# Autodesk Inventor assembly: ShredderImperial
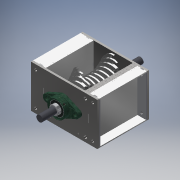
[picture p0: Inventor's stored thumbnail of the model, 180x180]
Saved by Autodesk Inventor 2018 (Build 220112000, 112)
## iProperties
Created: 2018-01-25
Part Number: ShredderImperial
Document SubType Name: Assembly
Designer: Olivier
Author: Olivier
## Documents named in this file (20)
- C:\Users\Olivier\OneDrive\Proyectos Olivier\Proyecto Shredder\Conversión Imperial\Inventor\Shredder Imperial\Autodesk Inventor 2018 files\ShredderImperial.iam
- C:\Users\Olivier\OneDrive\Proyectos Olivier\Proyecto Shredder\Conversión Imperial\Inventor\Shredder Imperial\Autodesk Inventor 2018 files\1-4inch_SidePanel_2-Parts.ipt
- C:\Users\Olivier\OneDrive\Proyectos Olivier\Proyecto Shredder\Conversión Imperial\Inventor\Shredder Imperial\Autodesk Inventor 2018 files\snr_ucfl204_0.ipt
- C:\Users\Olivier\OneDrive\Proyectos Olivier\Proyecto Shredder\Conversión Imperial\Inventor\Shredder Imperial\Autodesk Inventor 2018 files\HexBar1Inch.ipt
- C:\Users\Olivier\OneDrive\Proyectos Olivier\Proyecto Shredder\Conversión Imperial\Inventor\Shredder Imperial\Autodesk Inventor 2018 files\1-4inch_BearingSpacer_2-Parts.ipt
- C:\Users\Olivier\OneDrive\Proyectos Olivier\Proyecto Shredder\Conversión Imperial\Inventor\Shredder Imperial\Autodesk Inventor 2018 files\1-8inch_BearingSpacer_2-Parts.ipt
- C:\Users\Olivier\OneDrive\Proyectos Olivier\Proyecto Shredder\Conversión Imperial\Inventor\Shredder Imperial\Autodesk Inventor 2018 files\3-16inch_Knife1_5-Parts.ipt
- C:\Users\Olivier\OneDrive\Proyectos Olivier\Proyecto Shredder\Conversión Imperial\Inventor\Shredder Imperial\Autodesk Inventor 2018 files\3-16inch_Knife2_5-Parts.ipt
- C:\Users\Olivier\OneDrive\Proyectos Olivier\Proyecto Shredder\Conversión Imperial\Inventor\Shredder Imperial\Autodesk Inventor 2018 files\3-16inch_Knife3_4-Parts.ipt
- C:\Users\Olivier\OneDrive\Proyectos Olivier\Proyecto Shredder\Conversión Imperial\Inventor\Shredder Imperial\Autodesk Inventor 2018 files\1-4inch_KnifeSpacer_13-Parts.ipt
- C:\Users\Olivier\OneDrive\Proyectos Olivier\Proyecto Shredder\Conversión Imperial\Inventor\Shredder Imperial\Autodesk Inventor 2018 files\1-8inch_Sieve_2Parts.ipt
- C:\Users\Olivier\OneDrive\Proyectos Olivier\Proyecto Shredder\Conversión Imperial\Inventor\Shredder Imperial\Autodesk Inventor 2018 files\1-8inch_Side1_2-Parts.ipt
- C:\Users\Olivier\OneDrive\Proyectos Olivier\Proyecto Shredder\Conversión Imperial\Inventor\Shredder Imperial\Autodesk Inventor 2018 files\1-8inch_Side2_2-Parts.ipt
- C:\Users\Olivier\OneDrive\Proyectos Olivier\Proyecto Shredder\Conversión Imperial\Inventor\Shredder Imperial\Autodesk Inventor 2018 files\1-8inch_Top1_1-Part.ipt
- C:\Users\Olivier\OneDrive\Proyectos Olivier\Proyecto Shredder\Conversión Imperial\Inventor\Shredder Imperial\Autodesk Inventor 2018 files\1-8inch_Top2_1-Part.ipt
- C:\Users\Olivier\OneDrive\Proyectos Olivier\Proyecto Shredder\Conversión Imperial\Inventor\Shredder Imperial\Autodesk Inventor 2018 files\1-8inch_Bottom1_1-Part.ipt
- C:\Users\Olivier\OneDrive\Proyectos Olivier\Proyecto Shredder\Conversión Imperial\Inventor\Shredder Imperial\Autodesk Inventor 2018 files\1-8inch_Bottom2_1-Part.ipt
- C:\Users\Olivier\OneDrive\Proyectos Olivier\Proyecto Shredder\Conversión Imperial\Inventor\Shredder Imperial\Autodesk Inventor 2018 files\1-4inch_FixedKnifeSmall_14-Parts.ipt
- C:\Users\Olivier\OneDrive\Proyectos Olivier\Proyecto Shredder\Conversión Imperial\Inventor\Shredder Imperial\Autodesk Inventor 2018 files\3-16inch_FixedKnifeBig_13-Parts.ipt
- C:\Users\Olivier\OneDrive\Proyectos Olivier\Proyecto Shredder\Conversión Imperial\Inventor\Shredder Imperial\Autodesk Inventor 2018 files\1-8inch_Middle_2-Parts.ipt
## Components (75 placed, 19 different names)
1. 1-8inch_Middle_2-Parts:1 — Flush:18, Mate:233, Mate:234, Flush:20, Flush:21
2. 1-8inch_Middle_2-Parts:2 — Mate:225, Flush:14, Mate:226
3. 1-4inch_SidePanel_2-Parts:1 — Insert:1, Insert:2, Mate:96, Mate:97, Mate:120, Mate:121, Mate:123, Mate:215, Flush:13, Mate:222, Mate:223, Mate:224, Flush:15, Mate:230, Mate:231, Mate:232, Mate:233, Mate:235, Mate:236
4. 1-4inch_SidePanel_2-Parts:2 — Mate:91, Mate:92, Mate:93, Mate:94, Mate:95, Mate:203, Mate:204, Mate:207, Mate:218, Mate:219, Mate:220, Mate:225, Flush:14, Mate:227, Mate:228, Mate:229, Flush:16, Flush:18, Flush:19
5. 3-16inch_FixedKnifeBig_13-Parts:1 — Mate:122, Mate:124, Mate:125, Mate:126, Mate:127, Mate:128
6. 3-16inch_FixedKnifeBig_13-Parts:2 — Mate:129, Mate:130, Mate:131, Mate:132, Mate:133, Mate:134
7. 3-16inch_FixedKnifeBig_13-Parts:3 — Mate:135, Mate:136, Mate:137, Mate:138, Mate:139, Mate:140
8. 3-16inch_FixedKnifeBig_13-Parts:4 — Mate:141, Mate:142, Mate:143, Mate:144, Mate:145, Mate:146
9. 3-16inch_FixedKnifeBig_13-Parts:5 — Mate:147, Mate:148, Mate:149, Mate:150, Mate:151, Mate:152
10. 3-16inch_FixedKnifeBig_13-Parts:6 — Mate:153, Mate:154, Mate:155, Mate:156, Mate:157, Mate:158
11. 3-16inch_FixedKnifeBig_13-Parts:7 — Mate:159, Mate:160, Mate:161, Mate:162, Mate:163, Mate:164
12. 3-16inch_FixedKnifeBig_13-Parts:8 — Mate:165, Mate:166, Mate:167, Mate:168, Mate:169, Mate:170
13. 3-16inch_FixedKnifeBig_13-Parts:9 — Mate:171, Mate:172, Mate:173, Mate:174, Mate:175, Mate:176
14. 3-16inch_FixedKnifeBig_13-Parts:10 — Mate:177, Mate:178, Mate:179, Mate:180, Mate:181, Mate:182
15. 3-16inch_FixedKnifeBig_13-Parts:11 — Mate:183, Mate:184, Mate:185, Mate:186, Mate:187, Mate:188
16. 3-16inch_FixedKnifeBig_13-Parts:12 — Mate:189, Mate:190, Mate:191, Mate:192, Mate:193, Mate:194
17. 3-16inch_FixedKnifeBig_13-Parts:13 — Mate:195, Mate:196, Mate:197, Mate:198, Mate:199, Mate:200
18. 1-4inch_FixedKnifeSmall_14-Parts:1 — Mate:120, Mate:121, Mate:122, Mate:123, Mate:124, Mate:125, Mate:226
19. 1-4inch_FixedKnifeSmall_14-Parts:2 — Mate:126, Mate:127, Mate:128, Mate:129, Mate:130, Mate:131
20. 1-4inch_FixedKnifeSmall_14-Parts:3 — Mate:132, Mate:133, Mate:134, Mate:135, Mate:136, Mate:137
21. 1-4inch_FixedKnifeSmall_14-Parts:4 — Mate:138, Mate:139, Mate:140, Mate:141, Mate:142, Mate:143
22. 1-4inch_FixedKnifeSmall_14-Parts:5 — Mate:144, Mate:145, Mate:146, Mate:147, Mate:148, Mate:149
23. 1-4inch_FixedKnifeSmall_14-Parts:6 — Mate:150, Mate:151, Mate:152, Mate:153, Mate:154, Mate:155
24. 1-4inch_FixedKnifeSmall_14-Parts:7 — Mate:156, Mate:157, Mate:158, Mate:159, Mate:160, Mate:161
25. 1-4inch_FixedKnifeSmall_14-Parts:8 — Mate:162, Mate:163, Mate:164, Mate:165, Mate:166, Mate:167
26. 1-4inch_FixedKnifeSmall_14-Parts:9 — Mate:168, Mate:169, Mate:170, Mate:171, Mate:172, Mate:173
27. 1-4inch_FixedKnifeSmall_14-Parts:10 — Mate:174, Mate:175, Mate:176, Mate:177, Mate:178, Mate:179
28. 1-4inch_FixedKnifeSmall_14-Parts:11 — Mate:180, Mate:181, Mate:182, Mate:183, Mate:184, Mate:185
29. 1-4inch_FixedKnifeSmall_14-Parts:12 — Mate:186, Mate:187, Mate:188, Mate:189, Mate:190, Mate:191
30. 1-4inch_FixedKnifeSmall_14-Parts:13 — Mate:192, Mate:193, Mate:194, Mate:195, Mate:196, Mate:197
31. 1-4inch_FixedKnifeSmall_14-Parts:14 — Mate:198, Mate:199, Mate:200, Mate:203, Mate:204
32. HexBar1Inch:1 — Insert:3, Insert:4, Mate:5, Mate:6, Mate:7, Mate:9, Mate:10, Mate:11, Mate:12, Mate:13, Mate:15, Mate:16, Mate:17, Mate:18, Mate:21, Mate:22, Mate:23, Mate:24, Mate:27, Mate:28, Mate:30, Mate:31, Mate:33, Mate:34, Mate:36, Mate:37, Mate:39, Mate:40, Mate:42, Mate:43, Mate:45, Mate:46, Mate:48, Mate:49, Mate:51, Mate:52, Mate:54, Mate:55, Mate:57, Mate:58, Mate:60, Mate:61, Mate:63, Mate:64, Mate:66, Mate:67, Mate:69, Mate:70, Mate:71, Mate:72, Mate:75, Mate:76, Mate:78, Mate:79, Mate:80, Mate:82, Mate:83, Mate:85, Mate:86
33. snr_ucfl204_0:2 — Mate:91, Mate:92, Mate:93
34. snr_ucfl204_0:1 — Insert:1, Insert:2, Insert:7
35. 3-16inch_Knife1_5-Parts:1 — Mate:5, Mate:6, Mate:7, Mate:8
36. 3-16inch_Knife1_5-Parts:2 — Mate:21, Mate:22, Mate:26, Mate:29
37. 3-16inch_Knife1_5-Parts:3 — Mate:42, Mate:43, Mate:44, Mate:47
38. 3-16inch_Knife1_5-Parts:4 — Mate:60, Mate:61, Mate:62, Mate:65
39. 3-16inch_Knife1_5-Parts:5 — Mate:78, Mate:79, Mate:80, Mate:81, Mate:84
40. 3-16inch_Knife2_5-Parts:1 — Mate:12, Mate:13, Mate:14, Mate:19
41. 3-16inch_Knife2_5-Parts:2 — Mate:30, Mate:31, Mate:32, Mate:35
42. 3-16inch_Knife2_5-Parts:3 — Mate:48, Mate:49, Mate:50, Mate:53
43. 3-16inch_Knife2_5-Parts:4 — Mate:66, Mate:67, Mate:68, Mate:73
44. 3-16inch_Knife2_5-Parts:5 — Mate:85, Mate:86, Mate:87
45. 3-16inch_Knife3_4-Parts:1 — Mate:15, Mate:16, Mate:20, Mate:25
46. 3-16inch_Knife3_4-Parts:2 — Mate:36, Mate:37, Mate:38, Mate:41
47. 3-16inch_Knife3_4-Parts:3 — Mate:54, Mate:55, Mate:56, Mate:59
48. 3-16inch_Knife3_4-Parts:4 — Mate:69, Mate:70, Mate:74, Mate:77
49. 1-8inch_BearingSpacer_2-Parts:1 — Insert:3, Insert:5
50. 1-8inch_BearingSpacer_2-Parts:2 — Insert:4, Insert:6
51. 1-4inch_BearingSpacer_2-Parts:1 — Insert:5, Insert:7
52. 1-4inch_BearingSpacer_2-Parts:2 — Insert:6
53. 1-4inch_KnifeSpacer_13-Parts:1 — Mate:8, Mate:9, Mate:10, Mate:11, Mate:14
54. 1-4inch_KnifeSpacer_13-Parts:2 — Mate:17, Mate:18, Mate:19, Mate:20
55. 1-4inch_KnifeSpacer_13-Parts:3 — Mate:23, Mate:24, Mate:25, Mate:26
56. 1-4inch_KnifeSpacer_13-Parts:4 — Mate:27, Mate:28, Mate:29, Mate:32
57. 1-4inch_KnifeSpacer_13-Parts:5 — Mate:33, Mate:34, Mate:35, Mate:38
58. 1-4inch_KnifeSpacer_13-Parts:6 — Mate:39, Mate:40, Mate:41, Mate:44
59. 1-4inch_KnifeSpacer_13-Parts:7 — Mate:45, Mate:46, Mate:47, Mate:50
60. 1-4inch_KnifeSpacer_13-Parts:8 — Mate:51, Mate:52, Mate:53, Mate:56
61. 1-4inch_KnifeSpacer_13-Parts:9 — Mate:57, Mate:58, Mate:59, Mate:62
62. 1-4inch_KnifeSpacer_13-Parts:10 — Mate:63, Mate:64, Mate:65, Mate:68
63. 1-4inch_KnifeSpacer_13-Parts:11 — Mate:71, Mate:72, Mate:73, Mate:74
64. 1-4inch_KnifeSpacer_13-Parts:12 — Mate:75, Mate:76, Mate:77, Mate:81
65. 1-4inch_KnifeSpacer_13-Parts:13 — Mate:82, Mate:83, Mate:84, Mate:87
66. 1-8inch_Sieve_2Parts:2 — Mate:94, Mate:95
67. 1-8inch_Sieve_2Parts:1 — Mate:96, Mate:97
68. 1-8inch_Side1_2-Parts:1 — Mate:218, Mate:219, Mate:220
69. 1-8inch_Side1_2-Parts:2 — Mate:222, Mate:223, Mate:224
70. 1-8inch_Bottom1_1-Part:1 — Mate:215, Flush:13, Flush:15
71. 1-8inch_Top1_1-Part:1 — Mate:207
72. 1-8inch_Side2_2-Parts:1 — Mate:227, Mate:228, Mate:229
73. 1-8inch_Side2_2-Parts:2 — Mate:230, Mate:231, Mate:232, Mate:234
74. 1-8inch_Bottom2_1-Part:1 — Flush:16, Flush:21, Mate:236
75. 1-8inch_Top2_1-Part:1 — Flush:19, Mate:235, Flush:20
## Relationships (208: Mate 193, Flush 8, Insert 7)
- Insert:1: 1-4inch_SidePanel_2-Parts:1 ↔ snr_ucfl204_0:1
- Insert:2: 1-4inch_SidePanel_2-Parts:1 ↔ snr_ucfl204_0:1
- Insert:3: HexBar1Inch:1 ↔ 1-8inch_BearingSpacer_2-Parts:1
- Insert:4: HexBar1Inch:1 ↔ 1-8inch_BearingSpacer_2-Parts:2
- Insert:5: 1-8inch_BearingSpacer_2-Parts:1 ↔ 1-4inch_BearingSpacer_2-Parts:1
- Insert:6: 1-8inch_BearingSpacer_2-Parts:2 ↔ 1-4inch_BearingSpacer_2-Parts:2
- Insert:7: snr_ucfl204_0:1 ↔ 1-4inch_BearingSpacer_2-Parts:1
- Mate:5: HexBar1Inch:1 ↔ 3-16inch_Knife1_5-Parts:1
- Mate:6: HexBar1Inch:1 ↔ 3-16inch_Knife1_5-Parts:1
- Mate:7: HexBar1Inch:1 ↔ 3-16inch_Knife1_5-Parts:1
- Mate:8: 3-16inch_Knife1_5-Parts:1 ↔ 1-4inch_KnifeSpacer_13-Parts:1
- Mate:9: HexBar1Inch:1 ↔ 1-4inch_KnifeSpacer_13-Parts:1
- Mate:10: HexBar1Inch:1 ↔ 1-4inch_KnifeSpacer_13-Parts:1
- Mate:11: HexBar1Inch:1 ↔ 1-4inch_KnifeSpacer_13-Parts:1
- Mate:12: HexBar1Inch:1 ↔ 3-16inch_Knife2_5-Parts:1
- Mate:13: HexBar1Inch:1 ↔ 3-16inch_Knife2_5-Parts:1
- Mate:14: 3-16inch_Knife2_5-Parts:1 ↔ 1-4inch_KnifeSpacer_13-Parts:1
- Mate:15: HexBar1Inch:1 ↔ 3-16inch_Knife3_4-Parts:1
- Mate:16: HexBar1Inch:1 ↔ 3-16inch_Knife3_4-Parts:1
- Mate:17: HexBar1Inch:1 ↔ 1-4inch_KnifeSpacer_13-Parts:2
- Mate:18: HexBar1Inch:1 ↔ 1-4inch_KnifeSpacer_13-Parts:2
- Mate:19: 3-16inch_Knife2_5-Parts:1 ↔ 1-4inch_KnifeSpacer_13-Parts:2
- Mate:20: 3-16inch_Knife3_4-Parts:1 ↔ 1-4inch_KnifeSpacer_13-Parts:2
- Mate:21: HexBar1Inch:1 ↔ 3-16inch_Knife1_5-Parts:2
- Mate:22: HexBar1Inch:1 ↔ 3-16inch_Knife1_5-Parts:2
- Mate:23: HexBar1Inch:1 ↔ 1-4inch_KnifeSpacer_13-Parts:3
- Mate:24: HexBar1Inch:1 ↔ 1-4inch_KnifeSpacer_13-Parts:3
- Mate:25: 3-16inch_Knife3_4-Parts:1 ↔ 1-4inch_KnifeSpacer_13-Parts:3
- Mate:26: 3-16inch_Knife1_5-Parts:2 ↔ 1-4inch_KnifeSpacer_13-Parts:3
- Mate:27: HexBar1Inch:1 ↔ 1-4inch_KnifeSpacer_13-Parts:4
- Mate:28: HexBar1Inch:1 ↔ 1-4inch_KnifeSpacer_13-Parts:4
- Mate:29: 3-16inch_Knife1_5-Parts:2 ↔ 1-4inch_KnifeSpacer_13-Parts:4
- Mate:30: HexBar1Inch:1 ↔ 3-16inch_Knife2_5-Parts:2
- Mate:31: HexBar1Inch:1 ↔ 3-16inch_Knife2_5-Parts:2
- Mate:32: 3-16inch_Knife2_5-Parts:2 ↔ 1-4inch_KnifeSpacer_13-Parts:4
- Mate:33: HexBar1Inch:1 ↔ 1-4inch_KnifeSpacer_13-Parts:5
- Mate:34: HexBar1Inch:1 ↔ 1-4inch_KnifeSpacer_13-Parts:5
- Mate:35: 3-16inch_Knife2_5-Parts:2 ↔ 1-4inch_KnifeSpacer_13-Parts:5
- Mate:36: HexBar1Inch:1 ↔ 3-16inch_Knife3_4-Parts:2
- Mate:37: HexBar1Inch:1 ↔ 3-16inch_Knife3_4-Parts:2
- Mate:38: 3-16inch_Knife3_4-Parts:2 ↔ 1-4inch_KnifeSpacer_13-Parts:5
- Mate:39: HexBar1Inch:1 ↔ 1-4inch_KnifeSpacer_13-Parts:6
- Mate:40: HexBar1Inch:1 ↔ 1-4inch_KnifeSpacer_13-Parts:6
- Mate:41: 3-16inch_Knife3_4-Parts:2 ↔ 1-4inch_KnifeSpacer_13-Parts:6
- Mate:42: HexBar1Inch:1 ↔ 3-16inch_Knife1_5-Parts:3
- Mate:43: HexBar1Inch:1 ↔ 3-16inch_Knife1_5-Parts:3
- Mate:44: 3-16inch_Knife1_5-Parts:3 ↔ 1-4inch_KnifeSpacer_13-Parts:6
- Mate:45: HexBar1Inch:1 ↔ 1-4inch_KnifeSpacer_13-Parts:7
- Mate:46: HexBar1Inch:1 ↔ 1-4inch_KnifeSpacer_13-Parts:7
- Mate:47: 3-16inch_Knife1_5-Parts:3 ↔ 1-4inch_KnifeSpacer_13-Parts:7
- Mate:48: HexBar1Inch:1 ↔ 3-16inch_Knife2_5-Parts:3
- Mate:49: HexBar1Inch:1 ↔ 3-16inch_Knife2_5-Parts:3
- Mate:50: 3-16inch_Knife2_5-Parts:3 ↔ 1-4inch_KnifeSpacer_13-Parts:7
- Mate:51: HexBar1Inch:1 ↔ 1-4inch_KnifeSpacer_13-Parts:8
- Mate:52: HexBar1Inch:1 ↔ 1-4inch_KnifeSpacer_13-Parts:8
- Mate:53: 3-16inch_Knife2_5-Parts:3 ↔ 1-4inch_KnifeSpacer_13-Parts:8
- Mate:54: HexBar1Inch:1 ↔ 3-16inch_Knife3_4-Parts:3
- Mate:55: HexBar1Inch:1 ↔ 3-16inch_Knife3_4-Parts:3
- Mate:56: 3-16inch_Knife3_4-Parts:3 ↔ 1-4inch_KnifeSpacer_13-Parts:8
- Mate:57: HexBar1Inch:1 ↔ 1-4inch_KnifeSpacer_13-Parts:9
- Mate:58: HexBar1Inch:1 ↔ 1-4inch_KnifeSpacer_13-Parts:9
- Mate:59: 3-16inch_Knife3_4-Parts:3 ↔ 1-4inch_KnifeSpacer_13-Parts:9
- Mate:60: HexBar1Inch:1 ↔ 3-16inch_Knife1_5-Parts:4
- Mate:61: HexBar1Inch:1 ↔ 3-16inch_Knife1_5-Parts:4
- Mate:62: 3-16inch_Knife1_5-Parts:4 ↔ 1-4inch_KnifeSpacer_13-Parts:9
- Mate:63: HexBar1Inch:1 ↔ 1-4inch_KnifeSpacer_13-Parts:10
- Mate:64: HexBar1Inch:1 ↔ 1-4inch_KnifeSpacer_13-Parts:10
- Mate:65: 3-16inch_Knife1_5-Parts:4 ↔ 1-4inch_KnifeSpacer_13-Parts:10
- Mate:66: HexBar1Inch:1 ↔ 3-16inch_Knife2_5-Parts:4
- Mate:67: HexBar1Inch:1 ↔ 3-16inch_Knife2_5-Parts:4
- Mate:68: 3-16inch_Knife2_5-Parts:4 ↔ 1-4inch_KnifeSpacer_13-Parts:10
- Mate:69: HexBar1Inch:1 ↔ 3-16inch_Knife3_4-Parts:4
- Mate:70: HexBar1Inch:1 ↔ 3-16inch_Knife3_4-Parts:4
- Mate:71: HexBar1Inch:1 ↔ 1-4inch_KnifeSpacer_13-Parts:11
- Mate:72: HexBar1Inch:1 ↔ 1-4inch_KnifeSpacer_13-Parts:11
- Mate:73: 3-16inch_Knife2_5-Parts:4 ↔ 1-4inch_KnifeSpacer_13-Parts:11
- Mate:74: 3-16inch_Knife3_4-Parts:4 ↔ 1-4inch_KnifeSpacer_13-Parts:11
- Mate:75: HexBar1Inch:1 ↔ 1-4inch_KnifeSpacer_13-Parts:12
- Mate:76: HexBar1Inch:1 ↔ 1-4inch_KnifeSpacer_13-Parts:12
- Mate:77: 3-16inch_Knife3_4-Parts:4 ↔ 1-4inch_KnifeSpacer_13-Parts:12
- Mate:78: HexBar1Inch:1 ↔ 3-16inch_Knife1_5-Parts:5
- Mate:79: HexBar1Inch:1 ↔ 3-16inch_Knife1_5-Parts:5
- Mate:80: HexBar1Inch:1 ↔ 3-16inch_Knife1_5-Parts:5
- Mate:81: 3-16inch_Knife1_5-Parts:5 ↔ 1-4inch_KnifeSpacer_13-Parts:12
- Mate:82: HexBar1Inch:1 ↔ 1-4inch_KnifeSpacer_13-Parts:13
- Mate:83: HexBar1Inch:1 ↔ 1-4inch_KnifeSpacer_13-Parts:13
- Mate:84: 3-16inch_Knife1_5-Parts:5 ↔ 1-4inch_KnifeSpacer_13-Parts:13
- Mate:85: HexBar1Inch:1 ↔ 3-16inch_Knife2_5-Parts:5
- Mate:86: HexBar1Inch:1 ↔ 3-16inch_Knife2_5-Parts:5
- Mate:87: 3-16inch_Knife2_5-Parts:5 ↔ 1-4inch_KnifeSpacer_13-Parts:13
- Mate:91: 1-4inch_SidePanel_2-Parts:2 ↔ snr_ucfl204_0:2
- Mate:92: 1-4inch_SidePanel_2-Parts:2 ↔ snr_ucfl204_0:2
- Mate:93: 1-4inch_SidePanel_2-Parts:2 ↔ snr_ucfl204_0:2
- Mate:94: 1-4inch_SidePanel_2-Parts:2 ↔ 1-8inch_Sieve_2Parts:2
- Mate:95: 1-4inch_SidePanel_2-Parts:2 ↔ 1-8inch_Sieve_2Parts:2
- Mate:96: 1-4inch_SidePanel_2-Parts:1 ↔ 1-8inch_Sieve_2Parts:1
- Mate:97: 1-4inch_SidePanel_2-Parts:1 ↔ 1-8inch_Sieve_2Parts:1
- Mate:120: 1-4inch_SidePanel_2-Parts:1 ↔ 1-4inch_FixedKnifeSmall_14-Parts:1
- Mate:121: 1-4inch_SidePanel_2-Parts:1 ↔ 1-4inch_FixedKnifeSmall_14-Parts:1
- Mate:122: 3-16inch_FixedKnifeBig_13-Parts:1 ↔ 1-4inch_FixedKnifeSmall_14-Parts:1
- Mate:123: 1-4inch_SidePanel_2-Parts:1 ↔ 1-4inch_FixedKnifeSmall_14-Parts:1
- Mate:124: 3-16inch_FixedKnifeBig_13-Parts:1 ↔ 1-4inch_FixedKnifeSmall_14-Parts:1
- Mate:125: 3-16inch_FixedKnifeBig_13-Parts:1 ↔ 1-4inch_FixedKnifeSmall_14-Parts:1
- Mate:126: 3-16inch_FixedKnifeBig_13-Parts:1 ↔ 1-4inch_FixedKnifeSmall_14-Parts:2
- Mate:127: 3-16inch_FixedKnifeBig_13-Parts:1 ↔ 1-4inch_FixedKnifeSmall_14-Parts:2
- Mate:128: 3-16inch_FixedKnifeBig_13-Parts:1 ↔ 1-4inch_FixedKnifeSmall_14-Parts:2
- Mate:129: 3-16inch_FixedKnifeBig_13-Parts:2 ↔ 1-4inch_FixedKnifeSmall_14-Parts:2
- Mate:130: 3-16inch_FixedKnifeBig_13-Parts:2 ↔ 1-4inch_FixedKnifeSmall_14-Parts:2
- Mate:131: 3-16inch_FixedKnifeBig_13-Parts:2 ↔ 1-4inch_FixedKnifeSmall_14-Parts:2
- Mate:132: 3-16inch_FixedKnifeBig_13-Parts:2 ↔ 1-4inch_FixedKnifeSmall_14-Parts:3
- Mate:133: 3-16inch_FixedKnifeBig_13-Parts:2 ↔ 1-4inch_FixedKnifeSmall_14-Parts:3
- Mate:134: 3-16inch_FixedKnifeBig_13-Parts:2 ↔ 1-4inch_FixedKnifeSmall_14-Parts:3
- Mate:135: 3-16inch_FixedKnifeBig_13-Parts:3 ↔ 1-4inch_FixedKnifeSmall_14-Parts:3
- Mate:136: 3-16inch_FixedKnifeBig_13-Parts:3 ↔ 1-4inch_FixedKnifeSmall_14-Parts:3
- Mate:137: 3-16inch_FixedKnifeBig_13-Parts:3 ↔ 1-4inch_FixedKnifeSmall_14-Parts:3
- Mate:138: 3-16inch_FixedKnifeBig_13-Parts:3 ↔ 1-4inch_FixedKnifeSmall_14-Parts:4
- Mate:139: 3-16inch_FixedKnifeBig_13-Parts:3 ↔ 1-4inch_FixedKnifeSmall_14-Parts:4
- Mate:140: 3-16inch_FixedKnifeBig_13-Parts:3 ↔ 1-4inch_FixedKnifeSmall_14-Parts:4
- Mate:141: 3-16inch_FixedKnifeBig_13-Parts:4 ↔ 1-4inch_FixedKnifeSmall_14-Parts:4
- Mate:142: 3-16inch_FixedKnifeBig_13-Parts:4 ↔ 1-4inch_FixedKnifeSmall_14-Parts:4
- Mate:143: 3-16inch_FixedKnifeBig_13-Parts:4 ↔ 1-4inch_FixedKnifeSmall_14-Parts:4
- Mate:144: 3-16inch_FixedKnifeBig_13-Parts:4 ↔ 1-4inch_FixedKnifeSmall_14-Parts:5
- Mate:145: 3-16inch_FixedKnifeBig_13-Parts:4 ↔ 1-4inch_FixedKnifeSmall_14-Parts:5
- Mate:146: 3-16inch_FixedKnifeBig_13-Parts:4 ↔ 1-4inch_FixedKnifeSmall_14-Parts:5
- Mate:147: 3-16inch_FixedKnifeBig_13-Parts:5 ↔ 1-4inch_FixedKnifeSmall_14-Parts:5
- Mate:148: 3-16inch_FixedKnifeBig_13-Parts:5 ↔ 1-4inch_FixedKnifeSmall_14-Parts:5
- Mate:149: 3-16inch_FixedKnifeBig_13-Parts:5 ↔ 1-4inch_FixedKnifeSmall_14-Parts:5
- Mate:150: 3-16inch_FixedKnifeBig_13-Parts:5 ↔ 1-4inch_FixedKnifeSmall_14-Parts:6
- Mate:151: 3-16inch_FixedKnifeBig_13-Parts:5 ↔ 1-4inch_FixedKnifeSmall_14-Parts:6
- Mate:152: 3-16inch_FixedKnifeBig_13-Parts:5 ↔ 1-4inch_FixedKnifeSmall_14-Parts:6
- Mate:153: 3-16inch_FixedKnifeBig_13-Parts:6 ↔ 1-4inch_FixedKnifeSmall_14-Parts:6
- Mate:154: 3-16inch_FixedKnifeBig_13-Parts:6 ↔ 1-4inch_FixedKnifeSmall_14-Parts:6
- Mate:155: 3-16inch_FixedKnifeBig_13-Parts:6 ↔ 1-4inch_FixedKnifeSmall_14-Parts:6
- Mate:156: 3-16inch_FixedKnifeBig_13-Parts:6 ↔ 1-4inch_FixedKnifeSmall_14-Parts:7
- Mate:157: 3-16inch_FixedKnifeBig_13-Parts:6 ↔ 1-4inch_FixedKnifeSmall_14-Parts:7
- Mate:158: 3-16inch_FixedKnifeBig_13-Parts:6 ↔ 1-4inch_FixedKnifeSmall_14-Parts:7
- Mate:159: 3-16inch_FixedKnifeBig_13-Parts:7 ↔ 1-4inch_FixedKnifeSmall_14-Parts:7
- Mate:160: 3-16inch_FixedKnifeBig_13-Parts:7 ↔ 1-4inch_FixedKnifeSmall_14-Parts:7
- Mate:161: 3-16inch_FixedKnifeBig_13-Parts:7 ↔ 1-4inch_FixedKnifeSmall_14-Parts:7
- Mate:162: 3-16inch_FixedKnifeBig_13-Parts:7 ↔ 1-4inch_FixedKnifeSmall_14-Parts:8
- Mate:163: 3-16inch_FixedKnifeBig_13-Parts:7 ↔ 1-4inch_FixedKnifeSmall_14-Parts:8
- Mate:164: 3-16inch_FixedKnifeBig_13-Parts:7 ↔ 1-4inch_FixedKnifeSmall_14-Parts:8
- Mate:165: 3-16inch_FixedKnifeBig_13-Parts:8 ↔ 1-4inch_FixedKnifeSmall_14-Parts:8
- Mate:166: 3-16inch_FixedKnifeBig_13-Parts:8 ↔ 1-4inch_FixedKnifeSmall_14-Parts:8
- Mate:167: 3-16inch_FixedKnifeBig_13-Parts:8 ↔ 1-4inch_FixedKnifeSmall_14-Parts:8
- Mate:168: 3-16inch_FixedKnifeBig_13-Parts:8 ↔ 1-4inch_FixedKnifeSmall_14-Parts:9
- Mate:169: 3-16inch_FixedKnifeBig_13-Parts:8 ↔ 1-4inch_FixedKnifeSmall_14-Parts:9
- Mate:170: 3-16inch_FixedKnifeBig_13-Parts:8 ↔ 1-4inch_FixedKnifeSmall_14-Parts:9
- Mate:171: 3-16inch_FixedKnifeBig_13-Parts:9 ↔ 1-4inch_FixedKnifeSmall_14-Parts:9
- Mate:172: 3-16inch_FixedKnifeBig_13-Parts:9 ↔ 1-4inch_FixedKnifeSmall_14-Parts:9
- Mate:173: 3-16inch_FixedKnifeBig_13-Parts:9 ↔ 1-4inch_FixedKnifeSmall_14-Parts:9
- Mate:174: 3-16inch_FixedKnifeBig_13-Parts:9 ↔ 1-4inch_FixedKnifeSmall_14-Parts:10
- Mate:175: 3-16inch_FixedKnifeBig_13-Parts:9 ↔ 1-4inch_FixedKnifeSmall_14-Parts:10
- Mate:176: 3-16inch_FixedKnifeBig_13-Parts:9 ↔ 1-4inch_FixedKnifeSmall_14-Parts:10
- Mate:177: 3-16inch_FixedKnifeBig_13-Parts:10 ↔ 1-4inch_FixedKnifeSmall_14-Parts:10
- Mate:178: 3-16inch_FixedKnifeBig_13-Parts:10 ↔ 1-4inch_FixedKnifeSmall_14-Parts:10
- Mate:179: 3-16inch_FixedKnifeBig_13-Parts:10 ↔ 1-4inch_FixedKnifeSmall_14-Parts:10
- Mate:180: 3-16inch_FixedKnifeBig_13-Parts:10 ↔ 1-4inch_FixedKnifeSmall_14-Parts:11
- Mate:181: 3-16inch_FixedKnifeBig_13-Parts:10 ↔ 1-4inch_FixedKnifeSmall_14-Parts:11
- Mate:182: 3-16inch_FixedKnifeBig_13-Parts:10 ↔ 1-4inch_FixedKnifeSmall_14-Parts:11
- Mate:183: 3-16inch_FixedKnifeBig_13-Parts:11 ↔ 1-4inch_FixedKnifeSmall_14-Parts:11
- Mate:184: 3-16inch_FixedKnifeBig_13-Parts:11 ↔ 1-4inch_FixedKnifeSmall_14-Parts:11
- Mate:185: 3-16inch_FixedKnifeBig_13-Parts:11 ↔ 1-4inch_FixedKnifeSmall_14-Parts:11
- Mate:186: 3-16inch_FixedKnifeBig_13-Parts:11 ↔ 1-4inch_FixedKnifeSmall_14-Parts:12
- Mate:187: 3-16inch_FixedKnifeBig_13-Parts:11 ↔ 1-4inch_FixedKnifeSmall_14-Parts:12
- Mate:188: 3-16inch_FixedKnifeBig_13-Parts:11 ↔ 1-4inch_FixedKnifeSmall_14-Parts:12
- Mate:189: 3-16inch_FixedKnifeBig_13-Parts:12 ↔ 1-4inch_FixedKnifeSmall_14-Parts:12
- Mate:190: 3-16inch_FixedKnifeBig_13-Parts:12 ↔ 1-4inch_FixedKnifeSmall_14-Parts:12
- Mate:191: 3-16inch_FixedKnifeBig_13-Parts:12 ↔ 1-4inch_FixedKnifeSmall_14-Parts:12
- Mate:192: 3-16inch_FixedKnifeBig_13-Parts:12 ↔ 1-4inch_FixedKnifeSmall_14-Parts:13
- Mate:193: 3-16inch_FixedKnifeBig_13-Parts:12 ↔ 1-4inch_FixedKnifeSmall_14-Parts:13
- Mate:194: 3-16inch_FixedKnifeBig_13-Parts:12 ↔ 1-4inch_FixedKnifeSmall_14-Parts:13
- Mate:195: 3-16inch_FixedKnifeBig_13-Parts:13 ↔ 1-4inch_FixedKnifeSmall_14-Parts:13
- Mate:196: 3-16inch_FixedKnifeBig_13-Parts:13 ↔ 1-4inch_FixedKnifeSmall_14-Parts:13
- Mate:197: 3-16inch_FixedKnifeBig_13-Parts:13 ↔ 1-4inch_FixedKnifeSmall_14-Parts:13
- Mate:198: 3-16inch_FixedKnifeBig_13-Parts:13 ↔ 1-4inch_FixedKnifeSmall_14-Parts:14
- Mate:199: 3-16inch_FixedKnifeBig_13-Parts:13 ↔ 1-4inch_FixedKnifeSmall_14-Parts:14
- Mate:200: 3-16inch_FixedKnifeBig_13-Parts:13 ↔ 1-4inch_FixedKnifeSmall_14-Parts:14
- Mate:203: 1-4inch_SidePanel_2-Parts:2 ↔ 1-4inch_FixedKnifeSmall_14-Parts:14
- Mate:204: 1-4inch_SidePanel_2-Parts:2 ↔ 1-4inch_FixedKnifeSmall_14-Parts:14
- Mate:207: 1-4inch_SidePanel_2-Parts:2 ↔ 1-8inch_Top1_1-Part:1
- Mate:215: 1-4inch_SidePanel_2-Parts:1 ↔ 1-8inch_Bottom1_1-Part:1
- Flush:13: 1-4inch_SidePanel_2-Parts:1 ↔ 1-8inch_Bottom1_1-Part:1
- Mate:218: 1-4inch_SidePanel_2-Parts:2 ↔ 1-8inch_Side1_2-Parts:1
- Mate:219: 1-4inch_SidePanel_2-Parts:2 ↔ 1-8inch_Side1_2-Parts:1
- Mate:220: 1-4inch_SidePanel_2-Parts:2 ↔ 1-8inch_Side1_2-Parts:1
- Mate:222: 1-4inch_SidePanel_2-Parts:1 ↔ 1-8inch_Side1_2-Parts:2
- Mate:223: 1-4inch_SidePanel_2-Parts:1 ↔ 1-8inch_Side1_2-Parts:2
- Mate:224: 1-4inch_SidePanel_2-Parts:1 ↔ 1-8inch_Side1_2-Parts:2
- Mate:225: 1-8inch_Middle_2-Parts:2 ↔ 1-4inch_SidePanel_2-Parts:2
- Flush:14: 1-8inch_Middle_2-Parts:2 ↔ 1-4inch_SidePanel_2-Parts:2
- Mate:226: 1-8inch_Middle_2-Parts:2 ↔ 1-4inch_FixedKnifeSmall_14-Parts:1
- Flush:15: 1-4inch_SidePanel_2-Parts:1 ↔ 1-8inch_Bottom1_1-Part:1
- Mate:227: 1-4inch_SidePanel_2-Parts:2 ↔ 1-8inch_Side2_2-Parts:1
- Mate:228: 1-4inch_SidePanel_2-Parts:2 ↔ 1-8inch_Side2_2-Parts:1
- Mate:229: 1-4inch_SidePanel_2-Parts:2 ↔ 1-8inch_Side2_2-Parts:1
- Mate:230: 1-4inch_SidePanel_2-Parts:1 ↔ 1-8inch_Side2_2-Parts:2
- Mate:231: 1-4inch_SidePanel_2-Parts:1 ↔ 1-8inch_Side2_2-Parts:2
- Mate:232: 1-4inch_SidePanel_2-Parts:1 ↔ 1-8inch_Side2_2-Parts:2
- Flush:16: 1-4inch_SidePanel_2-Parts:2 ↔ 1-8inch_Bottom2_1-Part:1
- Flush:18: 1-8inch_Middle_2-Parts:1 ↔ 1-4inch_SidePanel_2-Parts:2
- Mate:233: 1-8inch_Middle_2-Parts:1 ↔ 1-4inch_SidePanel_2-Parts:1
- Mate:234: 1-8inch_Middle_2-Parts:1 ↔ 1-8inch_Side2_2-Parts:2
- Flush:19: 1-4inch_SidePanel_2-Parts:2 ↔ 1-8inch_Top2_1-Part:1
- Mate:235: 1-4inch_SidePanel_2-Parts:1 ↔ 1-8inch_Top2_1-Part:1
- Flush:20: 1-8inch_Middle_2-Parts:1 ↔ 1-8inch_Top2_1-Part:1
- Flush:21: 1-8inch_Middle_2-Parts:1 ↔ 1-8inch_Bottom2_1-Part:1
- Mate:236: 1-4inch_SidePanel_2-Parts:1 ↔ 1-8inch_Bottom2_1-Part:1
